# Autodesk Inventor assembly: Ensamble de Piezas
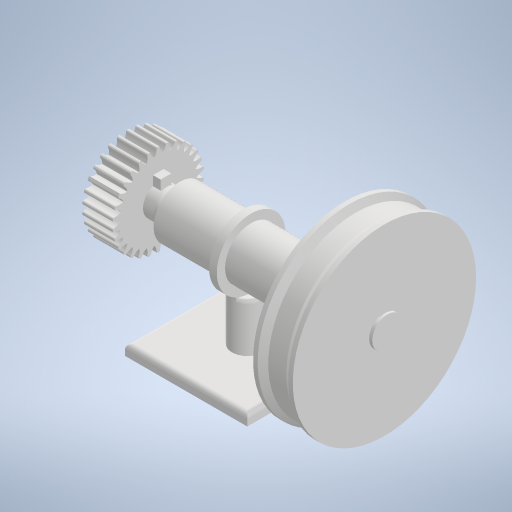
[picture p0: Inventor's stored thumbnail of the model, 512x512]
Saved by Autodesk Inventor 2024.2 (Build 282272000, 272)
## iProperties
Created: 2024-03-31
Part Number: Ensamble de Piezas
Document SubType Name: Assembly
Designer: Josh Juárez
Author: Josh Juárez
## Documents named in this file (6)
- D:\Universidad\Ciclo #5\Dinámica LAB\Tarea Ensamble\Ensamble de Piezas.iam
- D:\Universidad\Ciclo #5\Dinámica LAB\Tarea Ensamble\Piezas Otorgadas en Laboratorio\CUÑA.ipt
- D:\Universidad\Ciclo #5\Dinámica LAB\Tarea Ensamble\Piezas Otorgadas en Laboratorio\POLEA.ipt
- D:\Universidad\Ciclo #5\Dinámica LAB\Tarea Ensamble\Piezas Otorgadas en Laboratorio\ENGRANE.ipt
- D:\Universidad\Ciclo #5\Dinámica LAB\Tarea Ensamble\Piezas Otorgadas en Laboratorio\EJE_CUÑEROS.ipt
- D:\Universidad\Ciclo #5\Dinámica LAB\Tarea Ensamble\Nueva Pieza Realizada\Base para el Ensamble.ipt
## Components (6 placed, 5 different names)
1. POLEA:1 — Mate:2, Flush:1
2. ENGRANE:1 — Mate:1, Flush:2
3. EJE_CUÑEROS:1 — Rigid:1, Rigid:2, Mate:1, Mate:2, Mate:3
4. CUÑA:3 — Rigid:1, Flush:1
5. CUÑA:4 — Rigid:2, Flush:2
6. Base para el Ensamble:1 — Mate:3
## Relationships (7: Mate 3, WeldJoint 2, Flush 2)
- Rigid:1 [WeldJoint]: EJE_CUÑEROS:1 ↔ CUÑA:3
- Rigid:2 [WeldJoint]: EJE_CUÑEROS:1 ↔ CUÑA:4
- Mate:1: ENGRANE:1 ↔ EJE_CUÑEROS:1
- Mate:2: POLEA:1 ↔ EJE_CUÑEROS:1
- Flush:1: POLEA:1 ↔ CUÑA:3
- Mate:3: EJE_CUÑEROS:1 ↔ Base para el Ensamble:1
- Flush:2: ENGRANE:1 ↔ CUÑA:4
